# Autodesk Inventor assembly: L298N_motor_driver
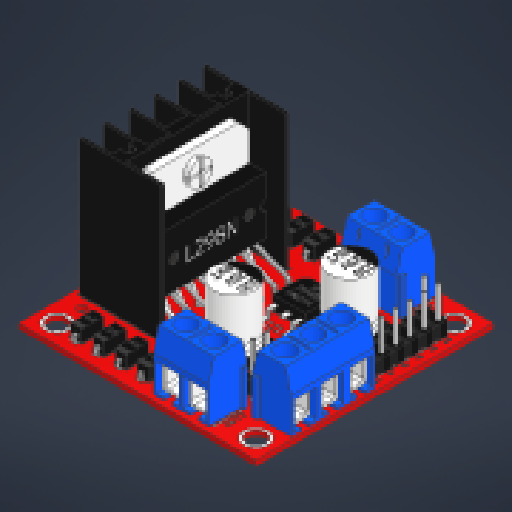
[picture p0: Inventor's stored thumbnail of the model, 512x512]
Saved by Autodesk Inventor 2026.1 (Build 301233020, 233B)
## iProperties
Created: 2025-11-26
Part Number: L298N_motor_driver
Document SubType Name: Assembly
Designer: jaewook
Author: jaewook
## Documents named in this file (3)
- C:\Users\kjh19\Documents\Inventor\project\final\base_device\L298N_motor_driver.iam
- C:\Users\kjh19\Downloads\motor-driver-l298n-3.snapshot.1\L298N.ipt
- C:\Users\kjh19\Documents\Inventor\project\final\base_device\L298N_base.ipt
## Components (2 placed, 2 different names)
1. L298N:1 — 강체:1
2. L298N_base:1 — 강체:1
## Relationships (1: WeldJoint 1)
- 강체:1 [WeldJoint]: L298N:1 ↔ L298N_base:1
